# Autodesk Inventor assembly: 36T_shaft
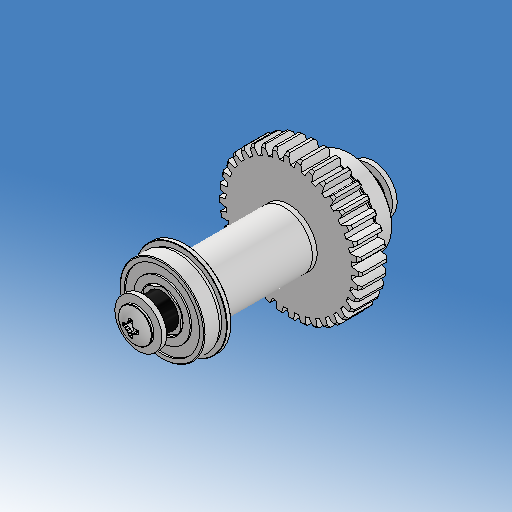
[picture p0: Inventor's stored thumbnail of the model, 512x512]
Saved by Autodesk Inventor 2025 (Build 290162000, 162)
## iProperties
Created: 2024-04-24
Part Number: 36T_shaft
Document SubType Name: Assembly
Designer: seene
Author: seene
## Documents named in this file (9)
- C:\Users\seene\OneDrive\SBRT\Robocup Rescue\Drive\v1\36T_shaft.iam
- C:\Users\seene\OneDrive\SBRT\Robocup Rescue\Drive\v1\REV-21-2813.ipt
- C:\Users\seene\OneDrive\SBRT\Robocup Rescue\Drive\v1\Gears\am-4709 36T 20DP 500hex 375 FW.ipt
- C:\Users\seene\OneDrive\SBRT\Robocup Rescue\Drive\v1\HexShaftSpacer.ipt
- C:\Users\seene\OneDrive\SBRT\Robocup Rescue\Drive\v1\REV-21-1916.ipt
- C:\Users\seene\OneDrive\SBRT\Robocup Rescue\Drive\v1\2879T1_High-Load Oil-Embedded 863 Bronze Thrust Bearing.ipt
- C:\Users\seene\OneDrive\SBRT\Robocup Rescue\Drive\v1\91770A830_Extra-Wide Truss Head Phillips Screws.ipt
- C:\Users\seene\OneDrive\SBRT\Robocup Rescue\Drive\v1\HexBearingDrivePlateSapcer.ipt
- C:\Users\seene\OneDrive\SBRT\Robocup Rescue\Drive\v1\am-3948-063 500H x 063IN Spacer.ipt
## Components (12 placed, 8 different names)
1. REV-21-2813:1 — Mate:5, Mate:8, Mate:10, Mate:12, Flush:1, Mate:23, Mate:24, Mate:26
2. am-4709 36T 20DP 500hex 375 FW:1 — Mate:5, Mate:13
3. HexShaftSpacer:1 — Mate:8, Mate:11
4. REV-21-1916:1 — Mate:10, Mate:11, Mate:14, Mate:25
5. REV-21-1916:2 — Mate:12, Mate:13, Mate:14, Flush:1, Mate:28
6. 2879T1_High-Load Oil-Embedded 863 Bronze Thrust Bearing:1 — Mate:15, Mate:16, Mate:18
7. 91770A830_Extra-Wide Truss Head Phillips Screws:1 — Mate:17, Mate:18
8. HexBearingDrivePlateSapcer:1 — Mate:15, Mate:16, Mate:17, Mate:24, Mate:26, Mate:27
9. 2879T1_High-Load Oil-Embedded 863 Bronze Thrust Bearing:2
10. 91770A830_Extra-Wide Truss Head Phillips Screws:2
11. HexBearingDrivePlateSapcer:2 — Mate:23, Mate:25
12. am-3948-063 500H x 063IN Spacer:1 — Mate:27, Mate:28
## Relationships (22: Mate 21, Flush 1)
- Mate:5: REV-21-2813:1 ↔ am-4709 36T 20DP 500hex 375 FW:1
- Mate:8: REV-21-2813:1 ↔ HexShaftSpacer:1
- Mate:10: REV-21-2813:1 ↔ REV-21-1916:1
- Mate:11: HexShaftSpacer:1 ↔ REV-21-1916:1
- Mate:12: REV-21-2813:1 ↔ REV-21-1916:2
- Mate:13 (1.5875 mm): am-4709 36T 20DP 500hex 375 FW:1 ↔ REV-21-1916:2
- Mate:14 (-50.8 mm): REV-21-1916:1 ↔ REV-21-1916:2
- Flush:1: REV-21-2813:1 ↔ REV-21-1916:2
- Mate:15: 2879T1_High-Load Oil-Embedded 863 Bronze Thrust Bearing:1 ↔ HexBearingDrivePlateSapcer:1
- Mate:16: 2879T1_High-Load Oil-Embedded 863 Bronze Thrust Bearing:1 ↔ HexBearingDrivePlateSapcer:1
- Mate:17: 91770A830_Extra-Wide Truss Head Phillips Screws:1 ↔ HexBearingDrivePlateSapcer:1
- Mate:18: 2879T1_High-Load Oil-Embedded 863 Bronze Thrust Bearing:1 ↔ 91770A830_Extra-Wide Truss Head Phillips Screws:1
- [Mate]: 2879T1_High-Load Oil-Embedded 863 Bronze Thrust Bearing:2 ↔ HexBearingDrivePlateSapcer:2
- [Mate]: 2879T1_High-Load Oil-Embedded 863 Bronze Thrust Bearing:2 ↔ HexBearingDrivePlateSapcer:2
- [Mate]: 91770A830_Extra-Wide Truss Head Phillips Screws:2 ↔ HexBearingDrivePlateSapcer:2
- [Mate]: 2879T1_High-Load Oil-Embedded 863 Bronze Thrust Bearing:2 ↔ 91770A830_Extra-Wide Truss Head Phillips Screws:2
- Mate:23: REV-21-2813:1 ↔ HexBearingDrivePlateSapcer:2
- Mate:24: REV-21-2813:1 ↔ HexBearingDrivePlateSapcer:1
- Mate:25: REV-21-1916:1 ↔ HexBearingDrivePlateSapcer:2
- Mate:26: REV-21-2813:1 ↔ HexBearingDrivePlateSapcer:1
- Mate:27: HexBearingDrivePlateSapcer:1 ↔ am-3948-063 500H x 063IN Spacer:1
- Mate:28: REV-21-1916:2 ↔ am-3948-063 500H x 063IN Spacer:1
## Named parameters: d25_d21 = 0 mm, d26_d22 = 0 mm, d27_d23 = 0 mm, d28_d24 = 0 mm
